# Autodesk Inventor assembly: 200-60-DIFFERENTIAL-CONNECTOR-01
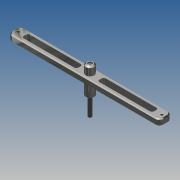
[picture p0: Inventor's stored thumbnail of the model, 180x180]
Saved by Autodesk Inventor 2018.2 (Build 222227000, 227)
## iProperties
Manager: feesmrt
Company: FRANC0R
Created: 2017-12-18
Part Number: 200-60-DIFFERENTIAL-CONNECTOR-01
Document SubType Name: Assembly
Designer: feesmrt
Project: Rescue Robot
Cost Center: -
Description: Differential Connector ASM
Engineer: feesmrt
Authority: feesmrt
Stock Number: 200-60-DIFFERENTIAL-CONNECTOR-01
Author: feesmrt
Title: Differential Connector ASM
Subject: Recue Robot
Revision Number: 1
## Documents named in this file (4)
- D:\Programmierung\FRANC0R\CAD\02-Rocker-Bogie-Robot\200-ROCKER-BOGIE\200-60-DIFFERENTIAL\200-60-DIFFERENTIAL-CONNECTOR-01.iam
- D:\Programmierung\FRANC0R\CAD\02-Rocker-Bogie-Robot\200-ROCKER-BOGIE\200-60-DIFFERENTIAL\200-60-DIFFERENTIAL-CONNECTOR-01.ipt
- D:\Programmierung\FRANC0R\CAD\02-Rocker-Bogie-Robot\200-ROCKER-BOGIE\200-60-DIFFERENTIAL\200-60-DIFFERENTIAL-CONNECTOR-02.ipt
- D:\Programmierung\FRANC0R\CAD\02-Rocker-Bogie-Robot\200-ROCKER-BOGIE\200-60-DIFFERENTIAL\200-60-DIFFERENTIAL-CONNECTOR-03.ipt
## Components (3 placed, 3 different names)
1. 200-60-DIFFERENTIAL-CONNECTOR-01:1 — Passend:1, Passend:2
2. 200-60-DIFFERENTIAL-CONNECTOR-02:1 — Passend:1, Passend:2, Passend:3, Passend:4
3. 200-60-DIFFERENTIAL-CONNECTOR-03:1 — Passend:3, Passend:4
## Relationships (4: Mate 4)
- Passend:1 [Mate]: 200-60-DIFFERENTIAL-CONNECTOR-01:1 ↔ 200-60-DIFFERENTIAL-CONNECTOR-02:1
- Passend:2 [Mate]: 200-60-DIFFERENTIAL-CONNECTOR-01:1 ↔ 200-60-DIFFERENTIAL-CONNECTOR-02:1
- Passend:3 [Mate]: 200-60-DIFFERENTIAL-CONNECTOR-02:1 ↔ 200-60-DIFFERENTIAL-CONNECTOR-03:1
- Passend:4 [Mate]: 200-60-DIFFERENTIAL-CONNECTOR-02:1 ↔ 200-60-DIFFERENTIAL-CONNECTOR-03:1
